# Autodesk Inventor assembly: neverest 40 + mounts + pulley + compliant wheel
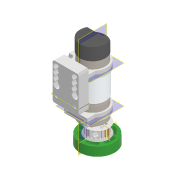
[picture p0: Inventor's stored thumbnail of the model, 180x180]
Saved by Autodesk Inventor 2020 (Build 240168000, 168)
## iProperties
Created: 2020-02-12
Part Number: neverest 40 + mounts + pulley + compliant wheel
Document SubType Name: Assembly
Designer: ball
Author: ball
## Documents named in this file (4)
- C:\FTC\FTC8863CAD\2019 Robot\Collection\neverest 40 + mounts + pulley + compliant wheel.iam
- C:\FTC\FTC8863CAD\2019 Robot\Collection\neverest 40 + mounts.iam
- C:\FTC\FTC8863CAD\2019 Robot\general robot componets\pulley .25 in + wheel.2.iam
- C:\FTC\FTC8863CAD\2019 Robot\Collection\intake motor mount to xrail fixed position.ipt
## Components (3 placed, 3 different names)
1. neverest 40 + mounts:1 [sub-assembly] — Mate:1, Mate:2, Mate:3, Angle:1, Mate:4
2. pulley .25 in + wheel.2:1 [sub-assembly] — Mate:1, Mate:2
3. intake motor mount to xrail fixed position:1 — Mate:3, Angle:1, Mate:4
## Relationships (5: Mate 4, Angle 1)
- Mate:1: neverest 40 + mounts:1 ↔ pulley .25 in + wheel.2:1
- Mate:2: neverest 40 + mounts:1 ↔ pulley .25 in + wheel.2:1
- Mate:3: neverest 40 + mounts:1 ↔ intake motor mount to xrail fixed position:1
- Angle:1 (0 deg): neverest 40 + mounts:1 ↔ intake motor mount to xrail fixed position:1
- Mate:4: neverest 40 + mounts:1 ↔ intake motor mount to xrail fixed position:1
